# Autodesk Inventor assembly: Weapon (Motor-Side Pulley)
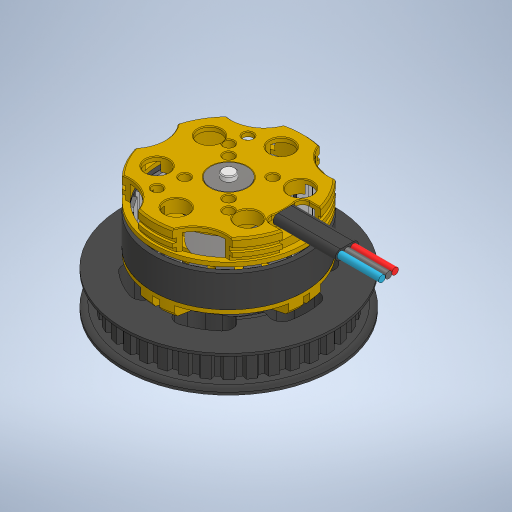
[picture p0: Inventor's stored thumbnail of the model, 512x512]
Saved by Autodesk Inventor 2023.2 (Build 272271000, 271)
## iProperties
Created: 2022-05-21
Part Number: Weapon (Motor-Side Pulley)
Document SubType Name: Assembly
Designer: Nathan Cai
Mass: 163.794 g
Surface Area: 513.523 cm^2
Volume: 53.858 cm^3
Density: 3.04123 g/cm^3
Author: Nathan Cai
## Documents named in this file (4)
- E:\Documents\Inventor\0.3rd Lawette - V3.5\Vertical Weapon Assembly (3rd Law)\Weapon (Motor-Side Pulley).iam
- E:\Documents\Inventor\0.3rd Lawette - V3.5\Vertical Weapon Assembly (3rd Law)\XL Pulley 36T .375in Wd.ipt
- E:\Documents\Inventor\0.3rd Lawette - V3.5\Vertical Weapon Assembly (3rd Law)\AeroSky_MC4822-390KV.ipt
- E:\Documents\Inventor\0.3rd Lawette - V3.5\Vertical Weapon Assembly (3rd Law)\FEICHAO BE4108 380KV\FEICHAO BE4108 380KV.iam
## Components (3 placed, 3 different names)
1. XL Pulley 36T .375in Wd:1 — Mate:2, Mate:3, Mate:4
2. AeroSky_MC4822-390KV:1 — Mate:2, Mate:3, Mate:4, Mate:5, Flush:1
3. FEICHAO BE4108 380KV:1 [sub-assembly] — Mate:5, Flush:1
## Relationships (5: Mate 4, Flush 1)
- Mate:2 (-34.925 mm): XL Pulley 36T .375in Wd:1 ↔ AeroSky_MC4822-390KV:1
- Mate:3: XL Pulley 36T .375in Wd:1 ↔ AeroSky_MC4822-390KV:1
- Mate:4: XL Pulley 36T .375in Wd:1 ↔ AeroSky_MC4822-390KV:1
- Mate:5: AeroSky_MC4822-390KV:1 ↔ FEICHAO BE4108 380KV:1
- Flush:1: AeroSky_MC4822-390KV:1 ↔ FEICHAO BE4108 380KV:1
